# Autodesk Inventor assembly: Assembly1
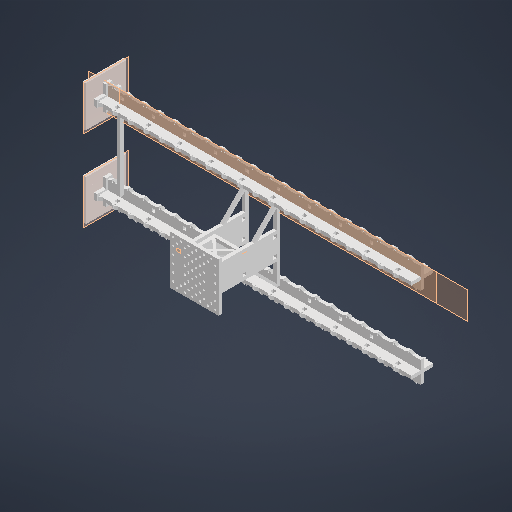
[picture p0: Inventor's stored thumbnail of the model, 512x512]
Saved by Autodesk Inventor 2027 (Build 310192000, 192)
## iProperties
Created: 2026-03-26
Part Number: Assembly1
Document SubType Name: Assembly
Designer: Tueha
Author: Tueha
## Documents named in this file (10)
- C:\Users\Tueha\OneDrive\Dokumenter\Inventor Files\Helix\Assembly1.iam
- C:\Users\Tueha\OneDrive\Dokumenter\Inventor Files\Helix\Bottom Body.ipt
- C:\Users\Tueha\OneDrive\Dokumenter\Inventor Files\Helix\TriangleConnector.ipt
- C:\Users\Tueha\OneDrive\Dokumenter\Inventor Files\Helix\Reflector.ipt
- C:\Users\Tueha\OneDrive\Dokumenter\Inventor Files\Helix\BetteKryds.ipt
- C:\Users\Tueha\OneDrive\Dokumenter\Inventor Files\Helix\ReinforcerLarge.ipt
- C:\Users\Tueha\OneDrive\Dokumenter\Inventor Files\Helix\FootTopLarge.ipt
- C:\Users\Tueha\OneDrive\Dokumenter\Inventor Files\Helix\ScrewPlateLarge.ipt
- C:\Users\Tueha\OneDrive\Dokumenter\Inventor Files\Helix\CrossReinforcement.ipt
- C:\Users\Tueha\OneDrive\Dokumenter\Inventor Files\Helix\CrossReinforcementUpper.ipt
## Components (16 placed, 9 different names)
1. ReinforcerLarge:1 — Flush:6
2. ScrewPlateLarge:1 — Flush:8
3. CrossReinforcement:1 — Flush:9
4. CrossReinforcementUpper:1 — Flush:10
5. Bottom Body:1 — Angle:1, Mate:1, Mate:2, Mate:3, Flush:3, Mate:5
6. Bottom Body:2 — Angle:1, Mate:1, Mate:2, Mate:3, Flush:2, Mate:4, Flush:6
7. TriangleConnector:1 — Flush:2, Flush:3, Mate:4
8. Reflector:1 — Mate:5, Flush:4, Flush:5
9. BetteKryds:1 — Flush:4, Flush:5
10. Bottom Body:3
11. Bottom Body:4 — Flush:7
12. TriangleConnector:2
13. Reflector:2
14. BetteKryds:2
15. FootTopLarge:1 — Flush:7, Flush:8, Flush:10
16. FootTopLarge:2 — Flush:9
## Component patterns: (2 elements, first: Bottom Body:1 + Bottom Body:2 + TriangleConnector:1 + Reflector:1 + BetteKryds:1), (2 elements, first: FootTopLarge:1)
## Relationships (15: Flush 9, Mate 5, Angle 1)
- Angle:1 (90 deg): Bottom Body:1 ↔ Bottom Body:2
- Mate:1: Bottom Body:1 ↔ Bottom Body:2
- Mate:2: Bottom Body:1 ↔ Bottom Body:2
- Mate:3: Bottom Body:1 ↔ Bottom Body:2
- Flush:2: Bottom Body:2 ↔ TriangleConnector:1
- Flush:3: Bottom Body:1 ↔ TriangleConnector:1
- Mate:4: Bottom Body:2 ↔ TriangleConnector:1
- Mate:5: Bottom Body:1 ↔ Reflector:1
- Flush:4: Reflector:1 ↔ BetteKryds:1
- Flush:5: Reflector:1 ↔ BetteKryds:1
- Flush:6: ReinforcerLarge:1 ↔ Bottom Body:2
- Flush:7: Bottom Body:4 ↔ FootTopLarge:1
- Flush:8: ScrewPlateLarge:1 ↔ FootTopLarge:1
- Flush:9: CrossReinforcement:1 ↔ FootTopLarge:2
- Flush:10: CrossReinforcementUpper:1 ↔ FootTopLarge:1
